# Autodesk Inventor assembly: Full Assembly Final
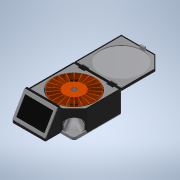
[picture p0: Inventor's stored thumbnail of the model, 180x180]
Saved by Autodesk Inventor 2022 (Build 260153000, 153)
## iProperties
Created: 2023-03-24
Part Number: Full Assembly Final
Document SubType Name: Assembly
Designer: zarek
Author: zarek
## Documents named in this file (4)
- C:\Users\zarek\OneDrive\Desktop\Random New Stuff\SPB\Full Assembly Final.iam
- C:\Users\zarek\OneDrive\Desktop\Random New Stuff\SPB\TouchScreen Housing\Touch Screen Assembly_2.iam
- C:\Users\zarek\OneDrive\Desktop\Random New Stuff\SPB\Overall Inside Assembly.iam
- C:\Users\zarek\OneDrive\Desktop\Random New Stuff\SPB\Lid Parts\Lid Assembly.iam
## Components (3 placed, 3 different names)
1. Touch Screen Assembly_2:1 [sub-assembly] — Rotational:1
2. Overall Inside Assembly:1 [sub-assembly] — Rotational:1, Flush:1, Mate:1
3. Lid Assembly:1 [sub-assembly] — Flush:1, Mate:1
## Relationships (3: RevoluteJoint 1, Flush 1, Mate 1)
- Rotational:1 [RevoluteJoint]: Touch Screen Assembly_2:1 ↔ Overall Inside Assembly:1
- Flush:1: Overall Inside Assembly:1 ↔ Lid Assembly:1
- Mate:1: Overall Inside Assembly:1 ↔ Lid Assembly:1
